# Autodesk Inventor assembly: płyta_bazowa_elewacji
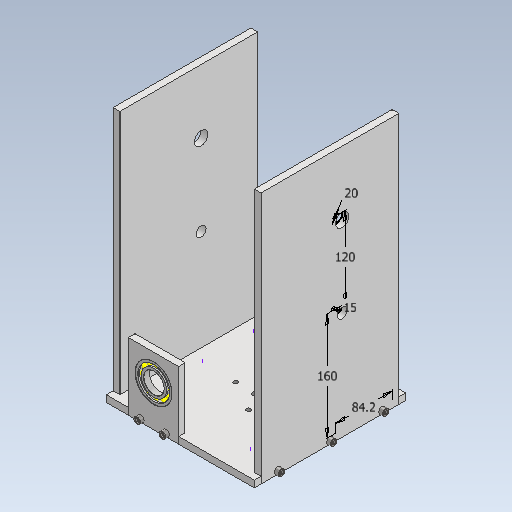
[picture p0: Inventor's stored thumbnail of the model, 512x512]
Saved by Autodesk Inventor 2020 (Build 240168000, 168)
## iProperties
Created: 2020-08-17
Part Number: płyta_bazowa_elewacji
Document SubType Name: Assembly
Designer: Hesekiel
Author: Hesekiel
## Documents named in this file (16)
- C:\Users\Hesekiel\Desktop\Equatorial-Mount-MUM\Mechanika\Mechanizm elewacji Filip\CAD\płyta_bazowa_elewacji.iam
- C:\Users\Hesekiel\Desktop\Equatorial-Mount-MUM\Mechanika\Mechanizm elewacji Filip\CAD\baza.ipt
- C:\Users\Hesekiel\Desktop\Equatorial-Mount-MUM\Mechanika\Mechanizm elewacji Filip\CAD\blok_łożyska.ipt
- C:\Users\Hesekiel\Desktop\Equatorial-Mount-MUM\Mechanika\Mechanizm elewacji Filip\CAD\płyta_bazowa_elewacji\Design Accelerator\Bolted Connection3.iam
- C:\Users\Hesekiel\Desktop\Equatorial-Mount-MUM\Mechanika\Mechanizm elewacji Filip\CAD\płyta_bazowa_elewacji\Design Accelerator\Bolted Connection4.iam
- C:\Users\Hesekiel\Desktop\Equatorial-Mount-MUM\Mechanika\Mechanizm elewacji Filip\CAD\płyta_bazowa_elewacji\Design Accelerator\Bolted Connection5.iam
- C:\Users\Hesekiel\Desktop\Equatorial-Mount-MUM\Mechanika\Mechanizm elewacji Filip\CAD\płyta_bazowa_elewacji\Design Accelerator\Bolted Connection6.iam
- C:\Users\Hesekiel\Desktop\Equatorial-Mount-MUM\Mechanika\Mechanizm elewacji Filip\CAD\płyta_boczna_obudowy.ipt
- C:\Users\Hesekiel\Desktop\Equatorial-Mount-MUM\Mechanika\Mechanizm elewacji Filip\CAD\płyta_bazowa_elewacji\Design Accelerator\Bolted Connection13.iam
- C:\Users\Hesekiel\Desktop\Equatorial-Mount-MUM\Mechanika\Mechanizm elewacji Filip\CAD\płyta_bazowa_elewacji\Design Accelerator\Bolted Connection14.iam
- C:\Users\Hesekiel\Desktop\Equatorial-Mount-MUM\Mechanika\Mechanizm elewacji Filip\CAD\płyta_bazowa_elewacji\Design Accelerator\Bolted Connection15.iam
- C:\Users\Hesekiel\Desktop\Equatorial-Mount-MUM\Mechanika\Mechanizm elewacji Filip\CAD\płyta_bazowa_elewacji\Design Accelerator\Bolted Connection16.iam
- C:\Users\Hesekiel\Desktop\Equatorial-Mount-MUM\Mechanika\Mechanizm elewacji Filip\CAD\płyta_bazowa_elewacji\Design Accelerator\Bolted Connection17.iam
- C:\Users\Hesekiel\Desktop\Equatorial-Mount-MUM\Mechanika\Mechanizm elewacji Filip\CAD\płyta_bazowa_elewacji\Design Accelerator\Bolted Connection18.iam
- C:\Users\Hesekiel\Desktop\Equatorial-Mount-MUM\Mechanika\Mechanizm elewacji Filip\CAD\SKF 16006\16006.iam
- C:\Users\Hesekiel\Desktop\Equatorial-Mount-MUM\Mechanika\Mechanizm elewacji Filip\CAD\płyta_boczna_obudowy_odbita.ipt
## Components (17 placed, 6 different names)
1. baza:1 — Mate:1, Mate:2, Mate:3, Mate:4, Mate:5, Mate:6, Flush:1, Mate:15, Mate:24, Mate:58, Flush:2, Mate:59
2. blok_łożyska:1 — Mate:4, Mate:5, Mate:6, Mate:48, Mate:49, Mate:50, Mate:51, Rigid:2
3. blok_łożyska:2 — Mate:1, Mate:2, Mate:3, Mate:44, Mate:45, Mate:46, Mate:47, Rigid:1
4. Bolted Connection:1 [sub-assembly] — Mate:44, Mate:45
5. Bolted Connection:2 [sub-assembly] — Mate:46, Mate:47
6. Bolted Connection:3 [sub-assembly] — Mate:48, Mate:49
7. Bolted Connection:4 [sub-assembly] — Mate:50, Mate:51
8. płyta_boczna_obudowy:1 — Flush:1, Mate:15, Mate:24, Mate:52, Mate:53, Mate:54, Mate:55, Mate:56, Mate:57
9. Bolted Connection:5 [sub-assembly] — Mate:52, Mate:53
10. Bolted Connection:6 [sub-assembly] — Mate:54, Mate:55
11. Bolted Connection:7 [sub-assembly] — Mate:56, Mate:57
12. Bolted Connection:8 [sub-assembly] — Mate:64, Mate:65
13. Bolted Connection:9 [sub-assembly] — Mate:62, Mate:63
14. Bolted Connection:10 [sub-assembly] — Mate:60, Mate:61
15. 16006:1 [sub-assembly] — Rigid:2
16. 16006:2 [sub-assembly] — Rigid:1
17. płyta_boczna_obudowy_odbita:1 — Mate:58, Flush:2, Mate:59, Mate:60, Mate:61, Mate:62, Mate:63, Mate:64, Mate:65
## Relationships (34: Mate 30, Flush 2, WeldJoint 2)
- Mate:1: baza:1 ↔ blok_łożyska:2
- Mate:2: baza:1 ↔ blok_łożyska:2
- Mate:3: baza:1 ↔ blok_łożyska:2
- Mate:4: baza:1 ↔ blok_łożyska:1
- Mate:5: baza:1 ↔ blok_łożyska:1
- Mate:6: baza:1 ↔ blok_łożyska:1
- Flush:1: baza:1 ↔ płyta_boczna_obudowy:1
- Mate:15: baza:1 ↔ płyta_boczna_obudowy:1
- Mate:24: baza:1 ↔ płyta_boczna_obudowy:1
- Mate:44: blok_łożyska:2 ↔ Bolted Connection:1
- Mate:45: blok_łożyska:2 ↔ Bolted Connection:1
- Mate:46: blok_łożyska:2 ↔ Bolted Connection:2
- Mate:47: blok_łożyska:2 ↔ Bolted Connection:2
- Mate:48: blok_łożyska:1 ↔ Bolted Connection:3
- Mate:49: blok_łożyska:1 ↔ Bolted Connection:3
- Mate:50: blok_łożyska:1 ↔ Bolted Connection:4
- Mate:51: blok_łożyska:1 ↔ Bolted Connection:4
- Mate:52: płyta_boczna_obudowy:1 ↔ Bolted Connection:5
- Mate:53: płyta_boczna_obudowy:1 ↔ Bolted Connection:5
- Mate:54: płyta_boczna_obudowy:1 ↔ Bolted Connection:6
- Mate:55: płyta_boczna_obudowy:1 ↔ Bolted Connection:6
- Mate:56: płyta_boczna_obudowy:1 ↔ Bolted Connection:7
- Mate:57: płyta_boczna_obudowy:1 ↔ Bolted Connection:7
- Rigid:1 [WeldJoint]: blok_łożyska:2 ↔ 16006:2
- Rigid:2 [WeldJoint]: blok_łożyska:1 ↔ 16006:1
- Mate:58: baza:1 ↔ płyta_boczna_obudowy_odbita:1
- Flush:2: baza:1 ↔ płyta_boczna_obudowy_odbita:1
- Mate:59: baza:1 ↔ płyta_boczna_obudowy_odbita:1
- Mate:60: Bolted Connection:10 ↔ płyta_boczna_obudowy_odbita:1
- Mate:61: Bolted Connection:10 ↔ płyta_boczna_obudowy_odbita:1
- Mate:62: Bolted Connection:9 ↔ płyta_boczna_obudowy_odbita:1
- Mate:63: Bolted Connection:9 ↔ płyta_boczna_obudowy_odbita:1
- Mate:64: Bolted Connection:8 ↔ płyta_boczna_obudowy_odbita:1
- Mate:65: Bolted Connection:8 ↔ płyta_boczna_obudowy_odbita:1
